# Autodesk Inventor assembly: left_leg
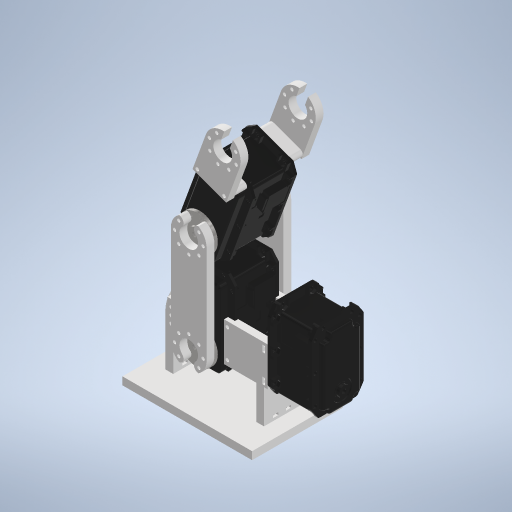
[picture p0: Inventor's stored thumbnail of the model, 512x512]
Saved by Autodesk Inventor 2024.3 (Build 283343000, 343)
## iProperties
Created: 2024-09-16
Part Number: left_leg
Document SubType Name: Assembly
Designer: USER
Author: USER
## Documents named in this file (12)
- C:\Users\USER\Desktop\로빛 예비인턴\(git)19기 이원준 격투로봇 설계파일\Lower_body\left_leg.iam
- C:\Users\USER\Desktop\로빛 예비인턴\(git)19기 이원준 격투로봇 설계파일\Lower_body\_foot.ipt
- C:\Users\USER\Desktop\로빛 예비인턴\(git)19기 이원준 격투로봇 설계파일\Lower_body\_foot_adt.ipt
- C:\Users\USER\Desktop\로빛 예비인턴\(git)19기 이원준 격투로봇 설계파일\motor\Motor_106.iam
- C:\Users\USER\Desktop\로빛 예비인턴\(git)19기 이원준 격투로봇 설계파일\Lower_body\_shim.ipt
- C:\Users\USER\Desktop\로빛 예비인턴\(git)19기 이원준 격투로봇 설계파일\Lower_body\_idle_adt.ipt
- C:\Users\USER\Desktop\로빛 예비인턴\(git)19기 이원준 격투로봇 설계파일\Lower_body\_adle_adt_2.ipt
- C:\Users\USER\Desktop\로빛 예비인턴\(git)19기 이원준 격투로봇 설계파일\아이들러\64아이들러.iam
- C:\Users\USER\Desktop\로빛 예비인턴\(git)19기 이원준 격투로봇 설계파일\motor\Motor_64_no_idle_ver.iam
- C:\Users\USER\Desktop\로빛 예비인턴\(git)19기 이원준 격투로봇 설계파일\Lower_body\_108-64_adt.ipt
- C:\Users\USER\Desktop\로빛 예비인턴\(git)19기 이원준 격투로봇 설계파일\Lower_body\_thigh.ipt
- C:\Users\USER\Desktop\로빛 예비인턴\(git)19기 이원준 격투로봇 설계파일\Lower_body\_thigh_2.ipt
## Components (18 placed, 11 different names)
1. _foot:2 — 메이트:2, 삽입:1, 삽입:2, 삽입:3, 삽입:4, 메이트:3, 각도:1
2. _foot_adt:1 — 삽입:1, 삽입:2, 삽입:11, 각도:3
3. _foot_adt:2 — 삽입:3, 삽입:4
4. _shim:2 — 플러쉬:1, 삽입:35, 삽입:36
5. _idle_adt:1 — 삽입:7, 삽입:8, 삽입:10
6. _adle_adt_2:1 — 삽입:5, 삽입:6, 삽입:7, 삽입:8, 삽입:12
7. _idle_adt:2 — 삽입:5, 삽입:6, 삽입:9
8. Motor_106:1 [sub-assembly] — 삽입:9, 삽입:10, 각도:1, 삽입:14, 삽입:15, 삽입:18, 삽입:19, 각도:2, 삽입:34, 삽입:35
9. 64아이들러:1 [sub-assembly] — 삽입:11, 삽입:12
10. Motor_64_no_idle_ver:1 [sub-assembly] — 삽입:16, 삽입:17, 삽입:20
11. _108-64_adt:1 — 삽입:18, 삽입:19, 삽입:20
12. _108-64_adt:2 — 삽입:14, 삽입:15, 삽입:16, 삽입:17
13. Motor_106:2 [sub-assembly] — 삽입:30, 삽입:31, 삽입:32, 삽입:33, 각도:2, 삽입:36
14. _thigh:1 — 삽입:26, 삽입:27, 삽입:32, 삽입:33
15. _thigh:2 — 삽입:28, 삽입:29, 삽입:30, 삽입:31
16. _thigh_2:1 — 삽입:26, 삽입:27
17. _thigh_2:2 — 삽입:28, 삽입:29
18. _shim:3 — 플러쉬:1, 각도:3, 삽입:34
## Relationships (36: Insert 30, Angle 3, Mate 2, Flush 1)
- 메이트:2 [Mate]: _foot:2
- 삽입:1 [Insert]: _foot:2 ↔ _foot_adt:1
- 삽입:2 [Insert]: _foot:2 ↔ _foot_adt:1
- 삽입:3 [Insert]: _foot:2 ↔ _foot_adt:2
- 삽입:4 [Insert]: _foot:2 ↔ _foot_adt:2
- 메이트:3 [Mate]: _foot:2
- 삽입:5 [Insert]: _adle_adt_2:1 ↔ _idle_adt:2
- 삽입:6 [Insert]: _adle_adt_2:1 ↔ _idle_adt:2
- 삽입:7 [Insert]: _idle_adt:1 ↔ _adle_adt_2:1
- 삽입:8 [Insert]: _idle_adt:1 ↔ _adle_adt_2:1
- 삽입:9 [Insert]: _idle_adt:2 ↔ Motor_106:1
- 삽입:10 [Insert]: _idle_adt:1 ↔ Motor_106:1
- 각도:1 [Angle] (0 deg): _foot:2 ↔ Motor_106:1
- 삽입:11 [Insert]: _foot_adt:1 ↔ 64아이들러:1
- 삽입:12 [Insert]: _adle_adt_2:1 ↔ 64아이들러:1
- 삽입:14 [Insert]: Motor_106:1 ↔ _108-64_adt:2
- 삽입:15 [Insert]: Motor_106:1 ↔ _108-64_adt:2
- 삽입:16 [Insert]: Motor_64_no_idle_ver:1 ↔ _108-64_adt:2
- 삽입:17 [Insert]: Motor_64_no_idle_ver:1 ↔ _108-64_adt:2
- 삽입:18 [Insert]: Motor_106:1 ↔ _108-64_adt:1
- 삽입:19 [Insert]: Motor_106:1 ↔ _108-64_adt:1
- 삽입:20 [Insert]: Motor_64_no_idle_ver:1 ↔ _108-64_adt:1
- 삽입:26 [Insert]: _thigh:1 ↔ _thigh_2:1
- 삽입:27 [Insert]: _thigh:1 ↔ _thigh_2:1
- 삽입:28 [Insert]: _thigh:2 ↔ _thigh_2:2
- 삽입:29 [Insert]: _thigh:2 ↔ _thigh_2:2
- 삽입:30 [Insert]: Motor_106:2 ↔ _thigh:2
- 삽입:31 [Insert]: Motor_106:2 ↔ _thigh:2
- 삽입:32 [Insert]: Motor_106:2 ↔ _thigh:1
- 삽입:33 [Insert]: Motor_106:2 ↔ _thigh:1
- 각도:2 [Angle] (-20 deg): Motor_106:1 ↔ Motor_106:2
- 플러쉬:1 [Flush]: _shim:2 ↔ _shim:3
- 각도:3 [Angle] (0 deg): _foot_adt:1 ↔ _shim:3
- 삽입:34 [Insert]: Motor_106:1 ↔ _shim:3
- 삽입:35 [Insert]: _shim:2 ↔ Motor_106:1
- 삽입:36 [Insert]: _shim:2 ↔ Motor_106:2
